# Autodesk Inventor assembly: Assembly1
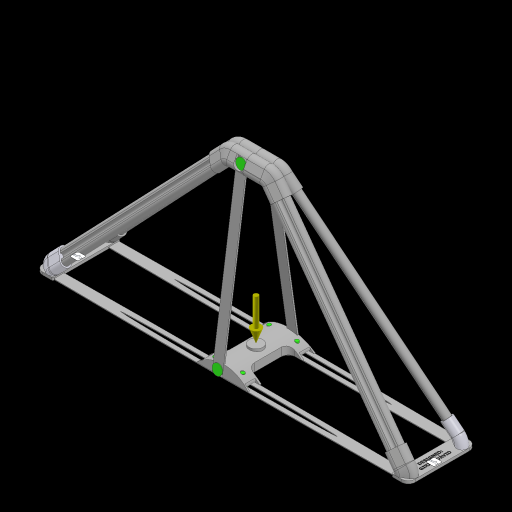
[picture p0: Inventor's stored thumbnail of the model, 512x512]
Saved by Autodesk Inventor 2023 (Build 270158000, 158)
## iProperties
Created: 2022-11-15
Part Number: Assembly1
Document SubType Name: Assembly
Designer: gd1
Author: gd1
## Documents named in this file (9)
- C:\Users\gd1\3D Objects\3D nagyteherbírású híd\Híd\H-d\Assembly1.iam
- C:\Users\gd1\3D Objects\3D nagyteherbírású híd\Híd\H-d\teljes6.iam
- C:\Users\gd1\3D Objects\3D nagyteherbírású híd\Híd\H-d\teljes5.iam
- C:\Users\gd1\3D Objects\3D nagyteherbírású híd\Híd\H-d\Assembly1\AIP\FEA\e5jv35dcw.fins
- C:\Users\gd1\3D Objects\3D nagyteherbírású híd\Híd\H-d\Assembly1\AIP\FEA\e5jv35dcw.fsat
- C:\Users\gd1\3D Objects\3D nagyteherbírású híd\Híd\H-d\Assembly1\AIP\FEA\e5jv35dcw.ftes
- C:\Users\gd1\3D Objects\3D nagyteherbírású híd\Híd\H-d\Assembly1\AIP\FEA\e5jv35dds.fwiz
- C:\Users\gd1\3D Objects\3D nagyteherbírású híd\Híd\H-d\Assembly1\AIP\FEA\e5jv35dy8.fmsh
- C:\Users\gd1\3D Objects\3D nagyteherbírású híd\Híd\H-d\Assembly1\AIP\FEA\e5jv35dy9.fres
## Components (2 placed, 2 different names)
1. teljes6:1 [sub-assembly] — Rigid:1
2. teljes5:1 [sub-assembly] — Rigid:1
## Relationships (1: WeldJoint 1)
- Rigid:1 [WeldJoint]: teljes6:1 ↔ teljes5:1
## Named parameters: sa_0 = 200000
note: some values were not read from the file. Shown as the stored number, unit unknown: "sa_0".
